# Autodesk Inventor assembly: ComederoV5
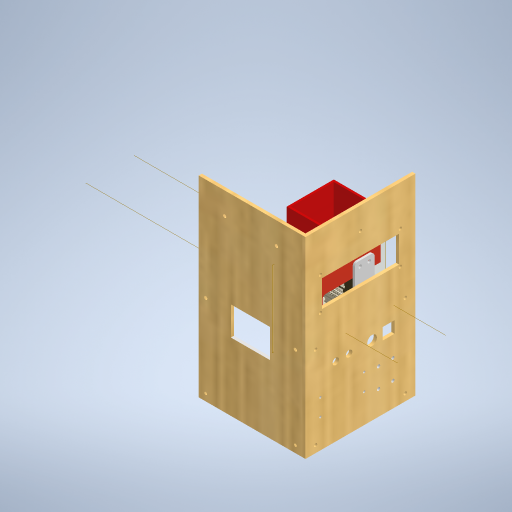
[picture p0: Inventor's stored thumbnail of the model, 512x512]
Saved by Autodesk Inventor 2023 (Build 270158000, 158)
## iProperties
Created: 2022-12-03
Part Number: ComederoV5
Document SubType Name: Assembly
Designer: sergi
Author: sergi
## Documents named in this file (15)
- C:\Users\sergi\OneDrive\Escritorio\Objetos 3d\ComederoV5\ComederoV5.iam
- C:\Users\sergi\OneDrive\Escritorio\Objetos 3d\ComederoV5\Panel1.ipt
- C:\Users\sergi\OneDrive\Escritorio\Objetos 3d\ComederoV5\Panel2.ipt
- C:\Users\sergi\OneDrive\Escritorio\Objetos 3d\ComederoV5\Panel3.ipt
- C:\Users\sergi\OneDrive\Escritorio\Objetos 3d\ComederoV5\Panel4.ipt
- C:\Users\sergi\OneDrive\Escritorio\Objetos 3d\ComederoV5\Tapa_abajo.ipt
- C:\Users\sergi\OneDrive\Escritorio\Objetos 3d\Rampa-Embudo.ipt
- C:\Users\sergi\OneDrive\Escritorio\Objetos 3d\Tolva1.ipt
- C:\Users\sergi\OneDrive\Escritorio\Objetos 3d\ComederoV5\Cinta.ipt
- C:\Users\sergi\OneDrive\Escritorio\Objetos 3d\ComederoV5\motor2.ipt
- C:\Users\sergi\OneDrive\Escritorio\Objetos 3d\Camisa Motor.ipt
- C:\Users\sergi\OneDrive\Escritorio\Objetos 3d\Rodillo2.ipt
- C:\Users\sergi\OneDrive\Escritorio\Objetos 3d\ComederoV5\ComederoV5\Design Accelerator\Transmisión de correas síncronas1.iam
- C:\Users\sergi\OneDrive\Escritorio\Objetos 3d\ComederoV5\cinta\Transmisión de correas síncronas1.iam
- C:\Users\sergi\OneDrive\Escritorio\Objetos 3d\ComederoV5\Soporte Motor2.ipt
## Components (14 placed, 13 different names)
1. Panel1:1 — Coincidencia:3, Nivelación:6, Nivelación:7, Nivelación:8, Coincidencia:6
2. Panel2:1 — Coincidencia:2, Nivelación:4, Nivelación:5, Coincidencia:3, Nivelación:6, Nivelación:9, Coincidencia:10, Coincidencia:13
3. Panel3:1 — Coincidencia:1, Nivelación:2, Nivelación:3, Nivelación:7, Coincidencia:4, Coincidencia:5, Coincidencia:7
4. Panel4:1 — Coincidencia:1, Nivelación:2, Nivelación:3, Coincidencia:2, Nivelación:4, Nivelación:5
5. Tapa_abajo:1 — Coincidencia:4, Nivelación:8, Nivelación:9
6. Rampa-Embudo:1 — Coincidencia:5, Coincidencia:6, Coincidencia:7, Nivelación:10, Coincidencia:8, Coincidencia:9
7. Tolva1:1 — Nivelación:10, Coincidencia:8, Coincidencia:9, Coincidencia:10, Coincidencia:11, Coincidencia:12, Coincidencia:14, Coincidencia:15, Coincidencia:17, Nivelación:16, Nivelación:17
8. Cinta:1 — Coincidencia:11, Coincidencia:12, Coincidencia:13, Nivelación:14
9. motor2:1 — Coincidencia:14, Coincidencia:15, Nivelación:11
10. Camisa Motor:1 — Nivelación:11, Nivelación:15
11. Rodillo2:1 — Nivelación:14, Nivelación:15, Coincidencia:16
12. Transmisión de correas síncronas:1 [sub-assembly]
13. Transmisión de correas síncronas:2 [sub-assembly] — Coincidencia:16, Coincidencia:17
14. Soporte Motor2:1 — Nivelación:16, Nivelación:17
## Relationships (31: Mate 17, Flush 14)
- Coincidencia:1 [Mate]: Panel3:1 ↔ Panel4:1
- Nivelación:2 [Flush]: Panel3:1 ↔ Panel4:1
- Nivelación:3 [Flush]: Panel3:1 ↔ Panel4:1
- Coincidencia:2 [Mate]: Panel2:1 ↔ Panel4:1
- Nivelación:4 [Flush]: Panel2:1 ↔ Panel4:1
- Nivelación:5 [Flush]: Panel2:1 ↔ Panel4:1
- Coincidencia:3 [Mate]: Panel1:1 ↔ Panel2:1
- Nivelación:6 [Flush]: Panel1:1 ↔ Panel2:1
- Nivelación:7 [Flush]: Panel1:1 ↔ Panel3:1
- Coincidencia:4 [Mate]: Panel3:1 ↔ Tapa_abajo:1
- Nivelación:8 [Flush]: Panel1:1 ↔ Tapa_abajo:1
- Nivelación:9 [Flush]: Panel2:1 ↔ Tapa_abajo:1
- Coincidencia:5 [Mate]: Panel3:1 ↔ Rampa-Embudo:1
- Coincidencia:6 [Mate]: Panel1:1 ↔ Rampa-Embudo:1
- Coincidencia:7 [Mate] (10 mm): Panel3:1 ↔ Rampa-Embudo:1
- Nivelación:10 [Flush]: Rampa-Embudo:1 ↔ Tolva1:1
- Coincidencia:8 [Mate]: Rampa-Embudo:1 ↔ Tolva1:1
- Coincidencia:9 [Mate]: Rampa-Embudo:1 ↔ Tolva1:1
- Coincidencia:10 [Mate]: Panel2:1 ↔ Tolva1:1
- Coincidencia:11 [Mate] (1 mm): Tolva1:1 ↔ Cinta:1
- Coincidencia:12 [Mate] (-4 mm): Tolva1:1 ↔ Cinta:1
- Coincidencia:13 [Mate] (17 mm): Panel2:1 ↔ Cinta:1
- Coincidencia:14 [Mate]: Tolva1:1 ↔ motor2:1
- Coincidencia:15 [Mate] (-2 mm): Tolva1:1 ↔ motor2:1
- Nivelación:11 [Flush]: motor2:1 ↔ Camisa Motor:1
- Nivelación:14 [Flush]: Cinta:1 ↔ Rodillo2:1
- Nivelación:15 [Flush] (2 mm): Camisa Motor:1 ↔ Rodillo2:1
- Coincidencia:16 [Mate]: Rodillo2:1 ↔ Transmisión de correas síncronas:2
- Coincidencia:17 [Mate]: Tolva1:1 ↔ Transmisión de correas síncronas:2
- Nivelación:16 [Flush]: Tolva1:1 ↔ Soporte Motor2:1
- Nivelación:17 [Flush]: Tolva1:1 ↔ Soporte Motor2:1
